# Autodesk Inventor assembly: 217-3195-200 Rev1
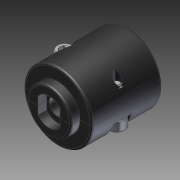
[picture p0: Inventor's stored thumbnail of the model, 180x180]
Saved by Autodesk Inventor 2014 SP1 (Build 180222100, 222)
## iProperties
Created: 2014-01-04
Part Number: 217-3195-200 Rev1
Document SubType Name: Assembly
Designer: Moses
Mass: 40.0223 g
Surface Area: 41.2275 cm^2
Volume: 5.09839 cm^3
Density: 7.85 g/cm^3
Author: Moses
## Documents named in this file (4)
- C:\Users\Moses\Documents\GitHub\2014buildCAD\chassisdrivetrain\gearbot\217-3433 (3 CIM Gearbox - WC)\217-3195-200 Rev1.iam
- C:\Users\Moses\Documents\GitHub\2014buildCAD\chassisdrivetrain\gearbot\217-3433 (3 CIM Gearbox - WC)\217-3195-010 Rev1.ipt
- C:\Users\Moses\Documents\GitHub\2014buildCAD\chassisdrivetrain\gearbot\217-3433 (3 CIM Gearbox - WC)\217-2778-NCQ8A075-050M_1032_Nut_90545A111.ipt
- C:\Users\Moses\Documents\GitHub\2014buildCAD\chassisdrivetrain\gearbot\217-3433 (3 CIM Gearbox - WC)\91251A107_91251A107.ipt
## Components (5 placed, 5 different names)
1. 217-3195-010 Rev1_82 — Mate:1, Flush:1, Mate:2, Insert:2, Mate:3, Mate:4, Angle:1
2. 217-3195-010 Rev1_83 — Mate:1, Flush:1, Mate:2, Insert:1
3. 217-2778-NCQ8A075-050M_1032_Nut_90545A111_84 — Mate:3, Mate:4, Angle:1
4. 91251A107_91251A107_85 — Insert:2
5. 91251A107_91251A107_86 — Insert:1
## Relationships (8: Mate 4, Insert 2, Flush 1, Angle 1)
- Mate:1: 217-3195-010 Rev1_82 ↔ 217-3195-010 Rev1_83
- Flush:1: 217-3195-010 Rev1_82 ↔ 217-3195-010 Rev1_83
- Mate:2: 217-3195-010 Rev1_82 ↔ 217-3195-010 Rev1_83
- Insert:1: 217-3195-010 Rev1_83 ↔ 91251A107_91251A107_86
- Insert:2: 217-3195-010 Rev1_82 ↔ 91251A107_91251A107_85
- Mate:3: 217-3195-010 Rev1_82 ↔ 217-2778-NCQ8A075-050M_1032_Nut_90545A111_84
- Mate:4: 217-3195-010 Rev1_82 ↔ 217-2778-NCQ8A075-050M_1032_Nut_90545A111_84
- Angle:1 (0 deg): 217-3195-010 Rev1_82 ↔ 217-2778-NCQ8A075-050M_1032_Nut_90545A111_84
